# Autodesk Inventor assembly: lukt_samsetning
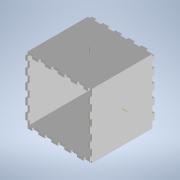
[picture p0: Inventor's stored thumbnail of the model, 180x180]
Saved by Autodesk Inventor 2021 (Build 250183000, 183)
## iProperties
Created: 2023-02-27
Part Number: lukt_samsetning
Document SubType Name: Assembly
Designer: frost
Author: frost
## Documents named in this file (2)
- C:\Users\frost\Velaverkfraedi\Vor - 2023\Tolvustud_framleidsla\lukt_samsetning.iam
- C:\Users\frost\Velaverkfraedi\Vor - 2023\Tolvustud_framleidsla\Lukt_hlidarplata.ipt
## Components (4 placed, 1 different names)
1. Lukt_hlidarplata:1 — Mate:1, Flush:1, Flush:2, Flush:3, Flush:4, Mate:2
2. Lukt_hlidarplata:2 — Flush:3, Flush:4, Mate:2, Flush:6
3. Lukt_hlidarplata:3 — Mate:1, Flush:1, Flush:2, Flush:7, Flush:8
4. Lukt_hlidarplata:4 — Flush:6, Flush:7, Flush:8
## Relationships (9: Flush 7, Mate 2)
- Mate:1: Lukt_hlidarplata:1 ↔ Lukt_hlidarplata:3
- Flush:1: Lukt_hlidarplata:1 ↔ Lukt_hlidarplata:3
- Flush:2: Lukt_hlidarplata:1 ↔ Lukt_hlidarplata:3
- Flush:3: Lukt_hlidarplata:1 ↔ Lukt_hlidarplata:2
- Flush:4: Lukt_hlidarplata:1 ↔ Lukt_hlidarplata:2
- Mate:2: Lukt_hlidarplata:1 ↔ Lukt_hlidarplata:2
- Flush:6: Lukt_hlidarplata:2 ↔ Lukt_hlidarplata:4
- Flush:7: Lukt_hlidarplata:3 ↔ Lukt_hlidarplata:4
- Flush:8: Lukt_hlidarplata:3 ↔ Lukt_hlidarplata:4
